# Autodesk Inventor assembly: Assembly2
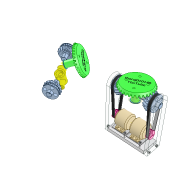
[picture p0: Inventor's stored thumbnail of the model, 180x180]
Saved by Autodesk Inventor 2022.5 (Build 265521000, 521)
## iProperties
Created: 2020-07-24
Part Number: Assembly2
Document SubType Name: Assembly
Designer: admin
Author: admin
## Documents named in this file (8)
- F:\YouTube\2024\YouTube\11N\9BevelGear2DoF\Assembly2E.iam
- F:\YouTube\2024\YouTube\11N\9BevelGear2DoF\B32x2i2.ipt
- F:\YouTube\2024\YouTube\11N\9BevelGear2DoF\B16x2i2.ipt
- F:\YouTube\2024\YouTube\11N\9BevelGear2DoF\Cross.ipt
- F:\YouTube\2024\YouTube\11N\9BevelGear2DoF\Pulley.ipt
- F:\YouTube\2024\YouTube\11N\9BevelGear2DoF\AssemblyFrame.iam
- F:\YouTube\2024\YouTube\11N\9BevelGear2DoF\Washer.ipt
- F:\YouTube\2024\YouTube\11N\9BevelGear2DoF\Bolt2W.ipt
## Components (17 placed, 7 different names)
1. AssemblyFrame:1 [sub-assembly] — Mate:1, Mate:2, Mate:3, Mate:4, Flush:1, Mate:5, Flush:2, Mate:8, Mate:9, Mate:11, Mate:10
2. Cross:1 — Mate:2, Mate:3, Mate:7, Mate:6
3. B32x2i2:1 — Mate:7, Mate:6, Insert:1
4. B16x2i2:1 — Mate:4, Flush:1
5. B16x2i2:2 — Mate:5, Flush:2
6. Pulley:1 — Mate:8, Mate:9
7. Pulley:2 — Mate:11, Mate:10
8. Washer:1 — Insert:1, Insert:2, Insert:3
9. Bolt2W:1 — Insert:2
10. Bolt2W:2 — Insert:3
11. Cross:2
12. B16x2i2:3
13. B16x2i2:4
14. B32x2i2:2
15. Washer:2
16. Bolt2W:3
17. Bolt2W:4
## Relationships (19: Mate 11, Insert 6, Flush 2)
- Mate:1: AssemblyFrame:1
- Mate:2 (20 mm): AssemblyFrame:1 ↔ Cross:1
- Mate:3: AssemblyFrame:1 ↔ Cross:1
- Mate:4: AssemblyFrame:1 ↔ B16x2i2:1
- Flush:1: AssemblyFrame:1 ↔ B16x2i2:1
- Mate:5: AssemblyFrame:1 ↔ B16x2i2:2
- Flush:2: AssemblyFrame:1 ↔ B16x2i2:2
- Mate:7: Cross:1 ↔ B32x2i2:1
- Mate:6: Cross:1 ↔ B32x2i2:1
- Mate:8: AssemblyFrame:1 ↔ Pulley:1
- Mate:9: AssemblyFrame:1 ↔ Pulley:1
- Mate:11: AssemblyFrame:1 ↔ Pulley:2
- Mate:10: AssemblyFrame:1 ↔ Pulley:2
- Insert:1: B32x2i2:1 ↔ Washer:1
- Insert:2: Washer:1 ↔ Bolt2W:1
- Insert:3: Washer:1 ↔ Bolt2W:2
- [Insert]: B32x2i2:2 ↔ Washer:2
- [Insert]: Washer:2 ↔ Bolt2W:3
- [Insert]: Washer:2 ↔ Bolt2W:4
## Named parameters: d113_d110 = 0 mm, d114_d111 = 0 mm, d115_d112 = 0 mm
